# Autodesk Inventor assembly: bosch four bar linkage
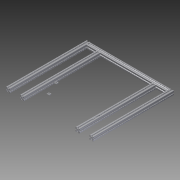
[picture p0: Inventor's stored thumbnail of the model, 180x180]
Saved by Autodesk Inventor 2013 (Build 170138000, 138)
## iProperties
Created: 2013-12-23
Part Number: bosch four bar linkage
Document SubType Name: Assembly
Designer: kahohbein
Author: kahohbein
## Documents named in this file (3)
- C:\Users\kahohbein\Documents\GitHub\2013-2014_BlockParty\CAD\bosch four bar linkage.iam
- C:\Users\kahohbein\Documents\GitHub\2013-2014_BlockParty\CAD\Drive\Final Drive Complete\Frame Layer open.iam
- C:\Users\kahohbein\Documents\GitHub\2013-2014_BlockParty\CAD\COTSParts\Bosch Extrusion\6mm block nut M4.ipt
## Components (5 placed, 2 different names)
1. Frame Layer open:1 [sub-assembly] — Mate:1, Mate:2, Mate:3, Mate:4
2. 6mm block nut M4:1
3. 6mm block nut M4:2
4. 6mm block nut M4:3 — Mate:3, Mate:4
5. 6mm block nut M4:4 — Mate:1, Mate:2
## Relationships (4: Mate 4)
- Mate:1: Frame Layer open:1 ↔ 6mm block nut M4:4
- Mate:2: Frame Layer open:1 ↔ 6mm block nut M4:4
- Mate:3: Frame Layer open:1 ↔ 6mm block nut M4:3
- Mate:4: Frame Layer open:1 ↔ 6mm block nut M4:3
